# Autodesk Inventor assembly: ASY ДМФ 101 кольцо со шпильками зад
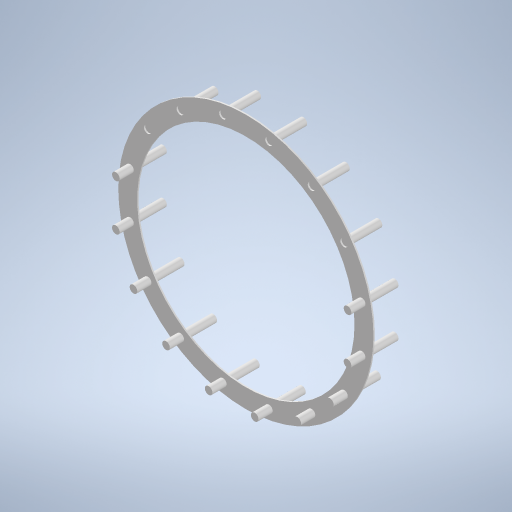
[picture p0: Inventor's stored thumbnail of the model, 512x512]
Saved by Autodesk Inventor 2024.2 (Build 282272000, 272)
## iProperties
Created: 2024-05-08
Part Number: ASY ДМФ 101 кольцо со шпильками зад
Document SubType Name: Assembly
Designer: pokla
Author: pokla
## Documents named in this file (5)
- C:\Users\admin\My Drive (bigstupidbeast@gmail.com)\Inventor\Disk Micro filter\DMF-Disk-Micro-Filter\ASY ДМФ 101 кольцо со шпильками зад.iam
- C:\Users\admin\My Drive (bigstupidbeast@gmail.com)\Inventor\Disk Micro filter\DMF-Disk-Micro-Filter\ДМС 011 кольцо под шпильки зад.ipt
- C:\Users\admin\My Drive (bigstupidbeast@gmail.com)\Inventor\Disk Micro filter\DMF-Disk-Micro-Filter\ДМС 030 шпилька 1.ipt
- C:\Users\admin\My Drive (bigstupidbeast@gmail.com)\Inventor\Disk Micro filter\DMF-Disk-Micro-Filter\ДМС 000 размеры.ipt
- C:\Users\admin\My Drive (bigstupidbeast@gmail.com)\Inventor\Disk Micro filter\DMF-Disk-Micro-Filter\ДМС 032 шпилька 2.ipt
## Components (17 placed, 3 different names)
1. ДМС 011 кольцо под шпильки зад:1 — Rigid:1, Rigid:2
2. ДМС 030 шпилька 1:1 — Rigid:1
3. ДМС 030 шпилька 1:2
4. ДМС 030 шпилька 1:3
5. ДМС 030 шпилька 1:4
6. ДМС 030 шпилька 1:5
7. ДМС 030 шпилька 1:6
8. ДМС 030 шпилька 1:7
9. ДМС 030 шпилька 1:8
10. ДМС 030 шпилька 1:9
11. ДМС 030 шпилька 1:10
12. ДМС 032 шпилька 2:1 — Rigid:2
13. ДМС 032 шпилька 2:2
14. ДМС 032 шпилька 2:3
15. ДМС 032 шпилька 2:4
16. ДМС 032 шпилька 2:5
17. ДМС 032 шпилька 2:6
## Component patterns: (10 elements, first: ДМС 030 шпилька 1:1), (6 elements, first: ДМС 032 шпилька 2:1)
## Relationships (2: WeldJoint 2)
- Rigid:1 [WeldJoint] (20 mm): ДМС 011 кольцо под шпильки зад:1 ↔ ДМС 030 шпилька 1:1
- Rigid:2 [WeldJoint]: ДМС 011 кольцо под шпильки зад:1 ↔ ДМС 032 шпилька 2:1
